# Autodesk Inventor assembly: MiniCybertruck
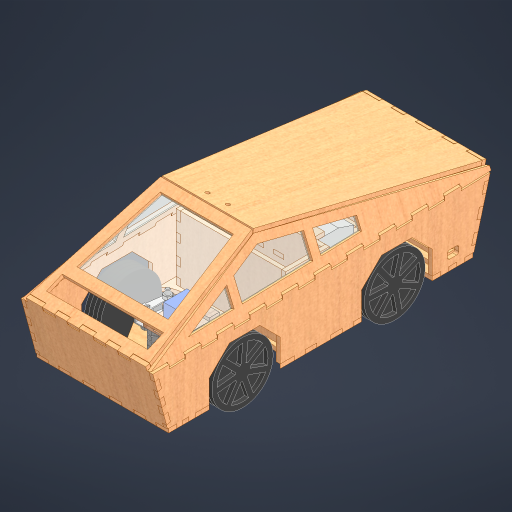
[picture p0: Inventor's stored thumbnail of the model, 512x512]
Saved by Autodesk Inventor 2023.2 (Build 272271000, 271)
## iProperties
Created: 2023-02-25
Part Number: MiniCybertruck
Document SubType Name: Assembly
Designer: natha
Author: natha
## Documents named in this file (37)
- C:\Users\natha\Documents\GitHub\Tesla-Mini\Other files\Inventor\MiniCybertruck.iam
- C:\Users\natha\Documents\GitHub\Tesla-Mini\Other files\Inventor\BottomPlate.ipt
- C:\Users\natha\Documents\GitHub\Tesla-Mini\Other files\Inventor\Motor.ipt
- C:\Users\natha\Documents\Inventor\Content Center Files\R2023\en-US\ANSI B18.6.7M(03)\ANSI B18.6.7M - M3x0.5 x 8(3).ipt
- C:\Users\natha\Documents\Inventor\Content Center Files\R2023\en-US\ANSI B 18.2.4.1 M(1)\ANSI B 18.2.4.1 M - M3 x 0.5Style 1.ipt
- C:\Users\natha\Documents\GitHub\Tesla-Mini\Other files\Inventor\FullWheelPlate.ipt
- C:\Users\natha\Documents\GitHub\Tesla-Mini\Other files\Inventor\WheelPlate_3mmHole.ipt
- C:\Users\natha\Documents\GitHub\Tesla-Mini\Other files\Inventor\TurnAxleHolder.ipt
- C:\Users\natha\Documents\Inventor\Content Center Files\R2023\en-US\ANSI B18.6.7M(03)\ANSI B18.6.7M - M4x0.7 x 20(3).ipt
- C:\Users\natha\Documents\Inventor\Content Center Files\R2023\en-US\ANSI B 18.2.4.1 M(1)\ANSI B 18.2.4.1 M - M4 x 0.7Style 1.ipt
- C:\Users\natha\Documents\GitHub\Tesla-Mini\Other files\Inventor\TurnAxleHolderConnector.ipt
- C:\Users\natha\Documents\GitHub\Tesla-Mini\Other files\Inventor\ServoBody.ipt
- C:\Users\natha\Documents\GitHub\Tesla-Mini\Other files\Inventor\ServoHead.ipt
- C:\Users\natha\Documents\Inventor\Content Center Files\R2023\en-US\JIS B 1111  H (2)\JIS B 1111 - A M2 x 8 - H(1).ipt
- C:\Users\natha\Documents\GitHub\Tesla-Mini\Other files\Inventor\ServoMountScrews.ipt
- C:\Users\natha\Documents\Inventor\Content Center Files\R2023\en-US\ISO 4032(2)\ISO 4032 - M5 - ISO.ipt
- C:\Users\natha\Documents\GitHub\Tesla-Mini\Other files\Inventor\ServoConnectorPin.ipt
- C:\Users\natha\Documents\Inventor\Content Center Files\R2023\en-US\ISO 4035(2)\ISO 4035 - M4 - ISO.ipt
- C:\Users\natha\Documents\GitHub\Tesla-Mini\Other files\Inventor\WheelPlate_4mmHole.ipt
- C:\Users\natha\Documents\GitHub\Tesla-Mini\Other files\Inventor\Phone.ipt
- C:\Users\natha\Documents\GitHub\Tesla-Mini\Other files\Inventor\BottomFrontplate.ipt
- C:\Users\natha\Documents\GitHub\Tesla-Mini\Other files\Inventor\BottomSidePlate.ipt
- C:\Users\natha\Documents\GitHub\Tesla-Mini\Other files\Inventor\BottomBackPlate.ipt
- C:\Users\natha\Documents\GitHub\Tesla-Mini\Other files\Inventor\TopSidePlate.ipt
- C:\Users\natha\Documents\GitHub\Tesla-Mini\Other files\Inventor\TopFrontPlate.ipt
- C:\Users\natha\Documents\GitHub\Tesla-Mini\Other files\Inventor\TopBackPlate.ipt
- C:\Users\natha\Documents\GitHub\Tesla-Mini\Other files\Inventor\PhoneHolder.ipt
- C:\Users\natha\Documents\GitHub\Tesla-Mini\Other files\Inventor\WeightContainerSide1.ipt
- C:\Users\natha\Documents\GitHub\Tesla-Mini\Other files\Inventor\WeightContainerSide2.ipt
- C:\Users\natha\Documents\GitHub\Tesla-Mini\Other files\Inventor\Pico.ipt
- C:\Users\natha\Documents\GitHub\Tesla-Mini\Other files\Inventor\PicoHolderBottom.ipt
- C:\Users\natha\Documents\GitHub\Tesla-Mini\Other files\Inventor\PicoHolderTop.ipt
- C:\Users\natha\Documents\GitHub\Tesla-Mini\Other files\Inventor\PicoNail.ipt
- C:\Users\natha\Documents\GitHub\Tesla-Mini\Other files\Inventor\LiftedPlate.ipt
- C:\Users\natha\Documents\GitHub\Tesla-Mini\Other files\Inventor\WeightContainerSide2Back.ipt
- C:\Users\natha\Documents\GitHub\Tesla-Mini\Other files\Inventor\TopFrontWindows.ipt
- C:\Users\natha\Documents\GitHub\Tesla-Mini\Other files\Inventor\TopSideWindows.ipt
## Components (89 placed, 36 different names)
1. BottomPlate:1 — Mate:1, Mate:2, Insert:33, Insert:34, Insert:39, Insert:40, Insert:64, Insert:65, Insert:66, Insert:67, Insert:84, Insert:85, Mate:8, Mate:9, Mate:13, Mate:14, Mate:29, Mate:30, Mate:32, Flush:1, Mate:38, Mate:39, Flush:2, Mate:40, Mate:41, Flush:3, Mate:42, Mate:43, Insert:121, Insert:122, Insert:123, Insert:124, Mate:47
2. Motor:1 — Insert:12, Insert:23, Insert:68, Insert:69, Insert:99
3. Slotted Pan Head Machine Screw - Metric M3x0.5 x 8:1
4. Slotted Pan Head Machine Screw - Metric M3x0.5 x 8:2 — Insert:33
5. Slotted Pan Head Machine Screw - Metric M3x0.5 x 8:3
6. Slotted Pan Head Machine Screw - Metric M3x0.5 x 8:4 — Insert:34
7. Hex Nut Metric M3 x 0.5:1 — Insert:65
8. Hex Nut Metric M3 x 0.5:2 — Insert:67, Insert:69
9. Hex Nut Metric M3 x 0.5:3 — Insert:64, Insert:68
10. Hex Nut Metric M3 x 0.5:4 — Insert:66
11. WheelPlate_3mmHole:1 — Insert:14
12. WheelPlate_3mmHole:2 — Insert:13, Insert:14
13. WheelPlate_3mmHole:3 — Insert:12, Insert:13, Insert:100
14. WheelPlate_3mmHole:4
15. WheelPlate_3mmHole:5
16. FullWheelPlate:4 — Insert:99
17. WheelPlate_3mmHole:6 — Insert:23
18. FullWheelPlate:5 — Insert:100
19. TurnAxleHolder:1 — Insert:35, Insert:37, Insert:41, Insert:43, Insert:44, Insert:87, Insert:96
20. TurnAxleHolder:2 — Insert:36, Insert:38, Insert:42, Insert:45, Insert:46, Insert:86, Insert:91
21. Slotted Pan Head Machine Screw - Metric M4x0.7 x 20:1 — Insert:36
22. Slotted Pan Head Machine Screw - Metric M4x0.7 x 20:2 — Insert:35
23. Hex Nut Metric M4 x 0.7:1 — Insert:38, Insert:39
24. Hex Nut Metric M4 x 0.7:2 — Insert:37, Insert:40
25. TurnAxleHolderConnector:1 — Insert:86, Insert:87, Tangent:1, Mate:6, Mate:7
26. Slotted Pan Head Machine Screw - Metric M4x0.7 x 20:3 — Insert:42
27. Slotted Pan Head Machine Screw - Metric M4x0.7 x 20:4 — Insert:41
28. Hex Nut Metric M4 x 0.7:3 — Insert:43
29. Hex Nut Metric M4 x 0.7:4 — Insert:44, Insert:89
30. Hex Nut Metric M4 x 0.7:5 — Insert:46
31. Hex Nut Metric M4 x 0.7:7 — Insert:45, Insert:88
32. FullWheelPlate:6 — Insert:97
33. WheelPlate_4mmHole:4
34. WheelPlate_4mmHole:5
35. WheelPlate_4mmHole:6 — Insert:96, Insert:97
36. FullWheelPlate:7 — Insert:98
37. WheelPlate_4mmHole:1 — Insert:91, Insert:92, Insert:98
38. WheelPlate_4mmHole:2 — Insert:92, Insert:93
39. WheelPlate_4mmHole:3 — Insert:93
40. ServoBody:1 — Insert:70, Insert:72, Insert:73, Insert:77, Insert:83
41. ServoHead:1 — Insert:70, Insert:71, Insert:90
42. JIS B 1111 H - Metric A M2 x 8 - H:1 — Insert:71
43. ServoMountScrews:1 — Insert:73
44. ServoMountScrews:2 — Insert:72
45. ISO 4032 M5:2 — Insert:74, Insert:84
46. ISO 4032 M5:3 — Insert:75, Insert:76
47. ISO 4032 M5:4 — Insert:74, Insert:75
48. ISO 4032 M5:5 — Insert:76, Insert:77
49. ISO 4032 M5:7 — Insert:85
50. ISO 4032 M5:8
51. ISO 4032 M5:9
52. ISO 4032 M5:10 — Insert:83
53. ServoConnectorPin:1 — Insert:90, Tangent:1, Mate:6, Mate:7
54. ISO 4035 M4:1 — Insert:88
55. ISO 4035 M4:2 — Insert:89
56. Phone:1 — Mate:28, Mate:31, Mate:32, Mate:33
57. BottomFrontplate:1 — Mate:10, Mate:11, Mate:15, Mate:26, Mate:27
58. BottomSidePlate:1 — Mate:8, Mate:9, Mate:10, Mate:11, Mate:18, Mate:19, Mate:20
59. BottomSidePlate:2 — Mate:13, Mate:14, Mate:15, Mate:16, Mate:17, Mate:21, Mate:22
60. BottomBackPlate:1 — Mate:16, Mate:17, Mate:18, Mate:24, Mate:25
61. TopSidePlate:1 — Mate:19, Mate:20, Mate:54, Mate:55
62. TopSidePlate:2 — Mate:21, Mate:22, Mate:52, Mate:53
63. TopFrontPlate:1 — Mate:26, Mate:27, Mate:28, Mate:33, Mate:50, Mate:51
64. TopBackPlate:1 — Mate:24, Mate:25
65. PhoneHolder:1 — Mate:29, Mate:30, Mate:31, Mate:34, Mate:35
66. PhoneHolder:2 — Mate:34, Mate:35, Mate:36, Mate:37
67. PhoneHolder:3 — Mate:36, Mate:37
68. WeightContainerSide1:1 — Flush:1, Mate:38, Mate:39, Flush:5
69. WeightContainerSide1:2 — Flush:2, Mate:40, Mate:41, Mate:46
70. WeightContainerSide2:1 — Flush:3, Mate:42, Mate:43
71. Pico:1 — Insert:105, Insert:106, Insert:109, Insert:110, Insert:111, Insert:112
72. PicoHolderBottom:1 — Insert:107, Insert:108, Insert:123, Insert:124
73. PicoHolderTop:1 — Insert:105, Insert:106, Insert:107, Insert:108
74. PicoNail:1 — Insert:109
75. PicoNail:2 — Insert:112
76. PicoNail:3 — Insert:111
77. PicoNail:4 — Insert:110
78. Pico:2
79. PicoHolderBottom:2 — Insert:121, Insert:122
80. PicoHolderTop:2
81. PicoNail:5
82. PicoNail:6
83. PicoNail:7
84. PicoNail:8
85. LiftedPlate:1 — Mate:48, Mate:49, Flush:6
86. WeightContainerSide2Back:1 — Mate:46, Mate:47, Flush:5, Mate:48, Mate:49, Flush:6
87. TopFrontWindows:1 — Mate:50, Mate:51
88. TopSideWindows:1 — Mate:54, Mate:55
89. TopSideWindows:2 — Mate:52, Mate:53
## Relationships (129: Insert 75, Mate 48, Flush 5, Tangent 1)
- Insert:12: Motor:1 ↔ WheelPlate_3mmHole:3
- Insert:13: WheelPlate_3mmHole:2 ↔ WheelPlate_3mmHole:3
- Insert:14: WheelPlate_3mmHole:1 ↔ WheelPlate_3mmHole:2
- Mate:1: BottomPlate:1
- Mate:2: BottomPlate:1
- [Insert]: WheelPlate_3mmHole:5 ↔ WheelPlate_3mmHole:6
- [Insert]: WheelPlate_3mmHole:4 ↔ WheelPlate_3mmHole:5
- Insert:23: Motor:1 ↔ WheelPlate_3mmHole:6
- Insert:33: BottomPlate:1 ↔ Slotted Pan Head Machine Screw - Metric M3x0.5 x 8:2
- Insert:34: BottomPlate:1 ↔ Slotted Pan Head Machine Screw - Metric M3x0.5 x 8:4
- Insert:35: TurnAxleHolder:1 ↔ Slotted Pan Head Machine Screw - Metric M4x0.7 x 20:2
- Insert:36: TurnAxleHolder:2 ↔ Slotted Pan Head Machine Screw - Metric M4x0.7 x 20:1
- Insert:37: TurnAxleHolder:1 ↔ Hex Nut Metric M4 x 0.7:2
- Insert:38: TurnAxleHolder:2 ↔ Hex Nut Metric M4 x 0.7:1
- Insert:39: BottomPlate:1 ↔ Hex Nut Metric M4 x 0.7:1
- Insert:40: BottomPlate:1 ↔ Hex Nut Metric M4 x 0.7:2
- Insert:41: TurnAxleHolder:1 ↔ Slotted Pan Head Machine Screw - Metric M4x0.7 x 20:4
- Insert:42: TurnAxleHolder:2 ↔ Slotted Pan Head Machine Screw - Metric M4x0.7 x 20:3
- Insert:43: TurnAxleHolder:1 ↔ Hex Nut Metric M4 x 0.7:3
- Insert:44: TurnAxleHolder:1 ↔ Hex Nut Metric M4 x 0.7:4
- Insert:45: TurnAxleHolder:2 ↔ Hex Nut Metric M4 x 0.7:7
- Insert:46: TurnAxleHolder:2 ↔ Hex Nut Metric M4 x 0.7:5
- Insert:64: BottomPlate:1 ↔ Hex Nut Metric M3 x 0.5:3
- Insert:65: BottomPlate:1 ↔ Hex Nut Metric M3 x 0.5:1
- Insert:66: BottomPlate:1 ↔ Hex Nut Metric M3 x 0.5:4
- Insert:67: BottomPlate:1 ↔ Hex Nut Metric M3 x 0.5:2
- Insert:68: Motor:1 ↔ Hex Nut Metric M3 x 0.5:3
- Insert:69: Motor:1 ↔ Hex Nut Metric M3 x 0.5:2
- Insert:70: ServoBody:1 ↔ ServoHead:1
- Insert:71: ServoHead:1 ↔ JIS B 1111 H - Metric A M2 x 8 - H:1
- Insert:72: ServoBody:1 ↔ ServoMountScrews:2
- Insert:73: ServoBody:1 ↔ ServoMountScrews:1
- Insert:74: ISO 4032 M5:2 ↔ ISO 4032 M5:4
- Insert:75: ISO 4032 M5:3 ↔ ISO 4032 M5:4
- Insert:76: ISO 4032 M5:3 ↔ ISO 4032 M5:5
- Insert:77: ServoBody:1 ↔ ISO 4032 M5:5
- [Insert]: ISO 4032 M5:7 ↔ ISO 4032 M5:9
- [Insert]: ISO 4032 M5:8 ↔ ISO 4032 M5:9
- [Insert]: ISO 4032 M5:8 ↔ ISO 4032 M5:10
- Insert:83: ServoBody:1 ↔ ISO 4032 M5:10
- Insert:84: BottomPlate:1 ↔ ISO 4032 M5:2
- Insert:85: BottomPlate:1 ↔ ISO 4032 M5:7
- Insert:86: TurnAxleHolder:2 ↔ TurnAxleHolderConnector:1
- Insert:87: TurnAxleHolder:1 ↔ TurnAxleHolderConnector:1
- Insert:88: Hex Nut Metric M4 x 0.7:7 ↔ ISO 4035 M4:1
- Insert:89: Hex Nut Metric M4 x 0.7:4 ↔ ISO 4035 M4:2
- Insert:90: ServoHead:1 ↔ ServoConnectorPin:1
- Tangent:1: TurnAxleHolderConnector:1 ↔ ServoConnectorPin:1
- Mate:6: TurnAxleHolderConnector:1 ↔ ServoConnectorPin:1
- Mate:7: TurnAxleHolderConnector:1 ↔ ServoConnectorPin:1
- Insert:91: TurnAxleHolder:2 ↔ WheelPlate_4mmHole:1
- Insert:92: WheelPlate_4mmHole:1 ↔ WheelPlate_4mmHole:2
- Insert:93: WheelPlate_4mmHole:2 ↔ WheelPlate_4mmHole:3
- [Insert]: WheelPlate_4mmHole:4 ↔ WheelPlate_4mmHole:5
- [Insert]: WheelPlate_4mmHole:5 ↔ WheelPlate_4mmHole:6
- Insert:96: TurnAxleHolder:1 ↔ WheelPlate_4mmHole:6
- Mate:8: BottomPlate:1 ↔ BottomSidePlate:1
- Mate:9: BottomPlate:1 ↔ BottomSidePlate:1
- Insert:97: FullWheelPlate:6 ↔ WheelPlate_4mmHole:6
- Insert:98: FullWheelPlate:7 ↔ WheelPlate_4mmHole:1
- Insert:99: Motor:1 ↔ FullWheelPlate:4
- Insert:100: WheelPlate_3mmHole:3 ↔ FullWheelPlate:5
- Mate:10: BottomFrontplate:1 ↔ BottomSidePlate:1
- Mate:11: BottomFrontplate:1 ↔ BottomSidePlate:1
- Mate:13: BottomPlate:1 ↔ BottomSidePlate:2
- Mate:14: BottomPlate:1 ↔ BottomSidePlate:2
- Mate:15: BottomFrontplate:1 ↔ BottomSidePlate:2
- Mate:16: BottomSidePlate:2 ↔ BottomBackPlate:1
- Mate:17: BottomSidePlate:2 ↔ BottomBackPlate:1
- Mate:18: BottomSidePlate:1 ↔ BottomBackPlate:1
- Mate:19: BottomSidePlate:1 ↔ TopSidePlate:1
- Mate:20: BottomSidePlate:1 ↔ TopSidePlate:1
- Mate:21: BottomSidePlate:2 ↔ TopSidePlate:2
- Mate:22: BottomSidePlate:2 ↔ TopSidePlate:2
- Mate:24: BottomBackPlate:1 ↔ TopBackPlate:1
- Mate:25: BottomBackPlate:1 ↔ TopBackPlate:1
- Mate:26: BottomFrontplate:1 ↔ TopFrontPlate:1
- Mate:27: BottomFrontplate:1 ↔ TopFrontPlate:1
- Mate:28: Phone:1 ↔ TopFrontPlate:1
- Mate:29: BottomPlate:1 ↔ PhoneHolder:1
- Mate:30: BottomPlate:1 ↔ PhoneHolder:1
- Mate:31: Phone:1 ↔ PhoneHolder:1
- Mate:32: BottomPlate:1 ↔ Phone:1
- Mate:33 (10.922 mm): Phone:1 ↔ TopFrontPlate:1
- Mate:34: PhoneHolder:1 ↔ PhoneHolder:2
- Mate:35: PhoneHolder:1 ↔ PhoneHolder:2
- Mate:36: PhoneHolder:2 ↔ PhoneHolder:3
- Mate:37: PhoneHolder:2 ↔ PhoneHolder:3
- Flush:1: BottomPlate:1 ↔ WeightContainerSide1:1
- Mate:38: BottomPlate:1 ↔ WeightContainerSide1:1
- Mate:39: BottomPlate:1 ↔ WeightContainerSide1:1
- Flush:2: BottomPlate:1 ↔ WeightContainerSide1:2
- Mate:40: BottomPlate:1 ↔ WeightContainerSide1:2
- Mate:41: BottomPlate:1 ↔ WeightContainerSide1:2
- Flush:3: BottomPlate:1 ↔ WeightContainerSide2:1
- Mate:42: BottomPlate:1 ↔ WeightContainerSide2:1
- Mate:43: BottomPlate:1 ↔ WeightContainerSide2:1
- Insert:105: Pico:1 ↔ PicoHolderTop:1
- Insert:106: Pico:1 ↔ PicoHolderTop:1
- Insert:107: PicoHolderBottom:1 ↔ PicoHolderTop:1
- Insert:108: PicoHolderBottom:1 ↔ PicoHolderTop:1
- Insert:109: Pico:1 ↔ PicoNail:1
- Insert:110: Pico:1 ↔ PicoNail:4
- Insert:111: Pico:1 ↔ PicoNail:3
- Insert:112: Pico:1 ↔ PicoNail:2
- [Insert]: Pico:2 ↔ PicoHolderTop:2
- [Insert]: Pico:2 ↔ PicoHolderTop:2
- [Insert]: PicoHolderBottom:2 ↔ PicoHolderTop:2
- [Insert]: PicoHolderBottom:2 ↔ PicoHolderTop:2
- [Insert]: Pico:2 ↔ PicoNail:5
- [Insert]: Pico:2 ↔ PicoNail:8
- [Insert]: Pico:2 ↔ PicoNail:7
- [Insert]: Pico:2 ↔ PicoNail:6
- Insert:121: BottomPlate:1 ↔ PicoHolderBottom:2
- Insert:122: BottomPlate:1 ↔ PicoHolderBottom:2
- Insert:123: BottomPlate:1 ↔ PicoHolderBottom:1
- Insert:124: BottomPlate:1 ↔ PicoHolderBottom:1
- Mate:46: WeightContainerSide1:2 ↔ WeightContainerSide2Back:1
- Mate:47: BottomPlate:1 ↔ WeightContainerSide2Back:1
- Flush:5: WeightContainerSide1:1 ↔ WeightContainerSide2Back:1
- Mate:48: LiftedPlate:1 ↔ WeightContainerSide2Back:1
- Mate:49: LiftedPlate:1 ↔ WeightContainerSide2Back:1
- Flush:6: LiftedPlate:1 ↔ WeightContainerSide2Back:1
- Mate:50: TopFrontPlate:1 ↔ TopFrontWindows:1
- Mate:51: TopFrontPlate:1 ↔ TopFrontWindows:1
- Mate:52: TopSidePlate:2 ↔ TopSideWindows:2
- Mate:53: TopSidePlate:2 ↔ TopSideWindows:2
- Mate:54: TopSidePlate:1 ↔ TopSideWindows:1
- Mate:55: TopSidePlate:1 ↔ TopSideWindows:1
## Named parameters: d35_d20 = 0 mm, d36_d21 = 0 mm, d97_d91 = 0 mm, d98_d92 = 0 mm, d99_d93 = 0 mm, d129_d127 = 0 mm, d130_d128 = 0 mm, d240_d223 = 0 mm, d241_d225 = 0 mm, d242_d239 = 0 mm, d243_d226 = 0 mm, d244_d227 = 0 mm, d245_d236 = 0 mm, d246_d237 = 0 mm, d247_d238 = 0 mm
